# Autodesk Inventor assembly: MonteCarloM1.2
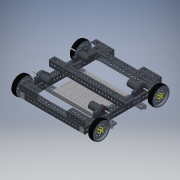
[picture p0: Inventor's stored thumbnail of the model, 180x180]
Saved by Autodesk Inventor 2016 (Build 200138000, 138)
## iProperties
Created: 2015-09-05
Part Number: MonteCarloM1.2
Document SubType Name: Assembly
Designer: Tim
Author: Tim
## Documents named in this file (7)
- C:\Users\Tim\Documents\GitHub\phi_robotics\3d-models\FTC_Tetrix_KOP_Block_Party\Tim Bloot Designs\MonteCarloM1.2.iam
- C:\Users\Tim\Documents\GitHub\phi_robotics\3d-models\FTC_Tetrix_KOP_Block_Party\Tim Bloot Designs\MonteCarloM1.1.iam
- C:\Users\Tim\Documents\GitHub\phi_robotics\3d-models\FTC_Tetrix_KOP_Block_Party\Tetrix_Kit_FTC\Autodesk Inventor Files\tetrix_motor_mount-old.ipt
- C:\Users\Tim\Documents\GitHub\phi_robotics\3d-models\FTC_Tetrix_KOP_Block_Party\Tetrix_Kit_FTC\Autodesk Inventor Files\tetrix_motor.iam
- C:\Users\Tim\Documents\GitHub\phi_robotics\3d-models\FTC_Tetrix_KOP_Block_Party\Tetrix_Kit_FTC\Autodesk Inventor Files\tetrix_c_channel-5.ipt
- C:\Users\Tim\Documents\GitHub\phi_robotics\3d-models\FTC_Tetrix_KOP_Block_Party\Tetrix_Kit_FTC\Autodesk Inventor Files\tetrix_c_channel-round.ipt
- C:\Users\Tim\Documents\GitHub\phi_robotics\3d-models\FTC_Tetrix_KOP_Block_Party\Tim Bloot Designs\MCPlate2.ipt
## Components (13 placed, 6 different names)
1. MonteCarloM1.1:1 [sub-assembly] — Rigid:1, Rigid:2, Rigid:3, Rigid:4, Rigid:7, Rigid:8, Rigid:9, Rigid:10
2. tetrix_motor_mount-old:1 — Rigid:3, Rotational:1
3. tetrix_motor_mount-old:2 — Rigid:1, Rotational:3
4. tetrix_motor_mount-old:3 — Rigid:2, Rotational:4
5. tetrix_motor_mount-old:4 — Rigid:4, Rotational:2
6. tetrix_motor:1 [sub-assembly] — Rotational:1
7. tetrix_motor:2 [sub-assembly] — Rotational:2
8. tetrix_motor:4 [sub-assembly] — Rotational:4
9. tetrix_motor:5 [sub-assembly] — Rotational:3
10. tetrix_c_channel-5:1
11. tetrix_c_channel-round:1 — Rigid:7
12. tetrix_c_channel-round:2 — Rigid:8
13. MCPlate2:1 — Rigid:9, Rigid:10
## Relationships (14: WeldJoint 10, RevoluteJoint 4)
- Rigid:1 [WeldJoint]: MonteCarloM1.1:1 ↔ tetrix_motor_mount-old:2
- Rigid:2 [WeldJoint]: MonteCarloM1.1:1 ↔ tetrix_motor_mount-old:3
- Rigid:3 [WeldJoint]: MonteCarloM1.1:1 ↔ tetrix_motor_mount-old:1
- Rigid:4 [WeldJoint]: MonteCarloM1.1:1 ↔ tetrix_motor_mount-old:4
- Rotational:1 [RevoluteJoint]: tetrix_motor_mount-old:1 ↔ tetrix_motor:1
- Rotational:2 [RevoluteJoint]: tetrix_motor_mount-old:4 ↔ tetrix_motor:2
- Rotational:3 [RevoluteJoint]: tetrix_motor_mount-old:2 ↔ tetrix_motor:5
- Rotational:4 [RevoluteJoint]: tetrix_motor_mount-old:3 ↔ tetrix_motor:4
- [WeldJoint]: tetrix_c_channel-5:1 ↔ tetrix_c_channel-round:1
- [WeldJoint]: tetrix_c_channel-5:1 ↔ tetrix_c_channel-round:2
- Rigid:7 [WeldJoint] (0.25 mm): MonteCarloM1.1:1 ↔ tetrix_c_channel-round:1
- Rigid:8 [WeldJoint] (0.25 mm): MonteCarloM1.1:1 ↔ tetrix_c_channel-round:2
- Rigid:9 [WeldJoint]: MonteCarloM1.1:1 ↔ MCPlate2:1
- Rigid:10 [WeldJoint]: MonteCarloM1.1:1 ↔ MCPlate2:1
